# Autodesk Inventor assembly: End_Effector
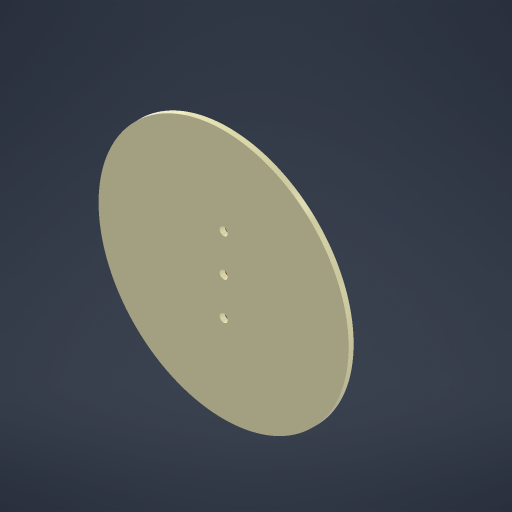
[picture p0: Inventor's stored thumbnail of the model, 512x512]
Saved by Autodesk Inventor 2023 (Build 270158000, 158)
## iProperties
Created: 2023-03-09
Part Number: End_Effector
Document SubType Name: Assembly
Designer: dzw04
Author: dzw04
## Documents named in this file (5)
- C:\Users\dzw04\Saxion\Mechatronica Lectoraat LMECH LED - Testomgeving van Dion\Component_Database\SAM2\01. Drawings\End_Effector\End_Effector.iam
- C:\Users\dzw04\Saxion\Mechatronica Lectoraat LMECH LED - Testomgeving van Dion\Component_Database\SAM2\01. Drawings\End_Effector\Base_V3.ipt
- C:\Users\dzw04\Saxion\Mechatronica Lectoraat LMECH LED - Testomgeving van Dion\Component_Database\SAM2\01. Drawings\End_Effector\Ball_v3.ipt
- C:\Users\dzw04\Saxion\Mechatronica Lectoraat LMECH LED - Testomgeving van Dion\Component_Database\SAM2\01. Drawings\End_Effector\Screw_V3.ipt
- C:\Users\dzw04\Saxion\Mechatronica Lectoraat LMECH LED - Testomgeving van Dion\Component_Database\SAM2\01. Drawings\End_Effector\Disc.ipt
## Components (4 placed, 4 different names)
1. Base_V3:1 — Ball:1, Mate:1, Mate:2
2. Ball_v3:1 — Ball:1, Mate:3, Mate:4
3. Screw_V3:1 — Mate:1, Mate:2
4. Disc:1 — Mate:3, Mate:4
## Relationships (5: Mate 4, BallJoint 1)
- Ball:1: Base_V3:1 ↔ Ball_v3:1
- Mate:1 (1 mm): Base_V3:1 ↔ Screw_V3:1
- Mate:2: Base_V3:1 ↔ Screw_V3:1
- Mate:3: Ball_v3:1 ↔ Disc:1
- Mate:4: Ball_v3:1 ↔ Disc:1
